# Autodesk Inventor assembly: 2022
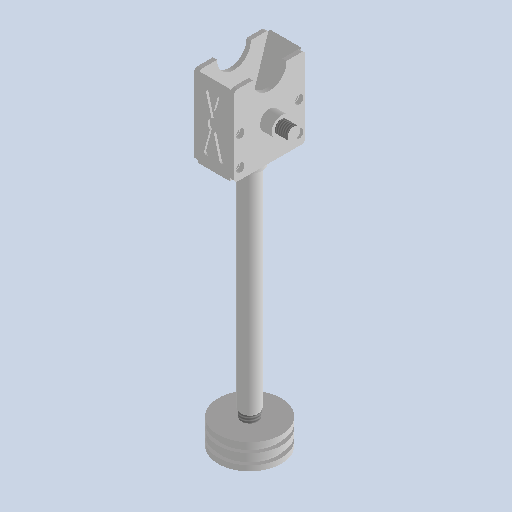
[picture p0: Inventor's stored thumbnail of the model, 512x512]
Saved by Autodesk Inventor 2025.1 (Build 291241000, 241)
## iProperties
Created: 2024-05-30
Part Number: 2022
Document SubType Name: Assembly
Designer: Fabri
Author: Fabri
## Documents named in this file (6)
- C:\Users\ffogue\Downloads\Meine Projket\Paddle\2022.iam
- C:\Users\ffogue\Downloads\Meine Projket\Paddle\2021.ipt
- C:\Users\ffogue\Downloads\Meine Projket\Paddle\2023.ipt
- C:\Users\ffogue\Downloads\Meine Projket\Paddle\blockAxis.ipt
- C:\Users\ffogue\Downloads\Meine Projket\Paddle\sheetblock.ipt
- C:\Users\ffogue\Downloads\Meine Projket\Paddle\2025.ipt
## Components (6 placed, 5 different names)
1. 2021:1 — Mate:4
2. 2023:1 — Mate:1, Mate:2, Insert:1, Insert:2, Mate:3, Insert:3
3. blockAxis:1 — Mate:3, Insert:3, Mate:4
4. sheetblock:1 — Mate:2, Insert:1
5. sheetblock:2 — Mate:1, Insert:2, Mate:5, Insert:5
6. 2025:1 — Mate:5, Insert:5
## Relationships (9: Mate 5, Insert 4)
- Mate:1: 2023:1 ↔ sheetblock:2
- Mate:2: 2023:1 ↔ sheetblock:1
- Insert:1: 2023:1 ↔ sheetblock:1
- Insert:2: 2023:1 ↔ sheetblock:2
- Mate:3: 2023:1 ↔ blockAxis:1
- Insert:3: 2023:1 ↔ blockAxis:1
- Mate:4: 2021:1 ↔ blockAxis:1
- Mate:5: sheetblock:2 ↔ 2025:1
- Insert:5: sheetblock:2 ↔ 2025:1
